# Autodesk Inventor assembly: Assembly1
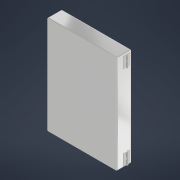
[picture p0: Inventor's stored thumbnail of the model, 180x180]
Saved by Autodesk Inventor 2022 (Build 260153000, 153)
## iProperties
Created: 2021-05-25
Part Number: Assembly1
Document SubType Name: Assembly
Designer: Albert L Tomberg
Mass: 5171.74 g
Surface Area: 5904.03 cm^2
Volume: 1915.46 cm^3
Density: 2.7 g/cm^3
Author: Albert L Tomberg
## Documents named in this file (4)
- C:\Users\Albert L Tomberg\Documents\CAD School\Assembly1.iam
- C:\Users\Albert L Tomberg\Documents\CAD School\Pocker lower half.ipt
- C:\Users\Albert L Tomberg\Documents\CAD School\Pocker higher half.ipt
- C:\Users\Albert L Tomberg\Documents\CAD School\Hinge.iam
## Components (4 placed, 3 different names)
1. Pocker lower half:1 — Mate:1, Mate:2, Mate:11, Mate:12, Mate:13
2. Pocker higher half:1 — Mate:4, Mate:6, Mate:7, Mate:8, Mate:12
3. Hinge:1 [sub-assembly] — Mate:4, Flush:1, Mate:7, Mate:11, Mate:13
4. Hinge:2 [sub-assembly] — Mate:6, Flush:1, Mate:8
## Relationships (10: Mate 9, Flush 1)
- Mate:1: Pocker lower half:1
- Mate:2: Pocker lower half:1
- Mate:4: Pocker higher half:1 ↔ Hinge:1
- Mate:6: Pocker higher half:1 ↔ Hinge:2
- Flush:1: Hinge:1 ↔ Hinge:2
- Mate:7: Pocker higher half:1 ↔ Hinge:1
- Mate:8: Pocker higher half:1 ↔ Hinge:2
- Mate:11: Pocker lower half:1 ↔ Hinge:1
- Mate:12: Pocker lower half:1 ↔ Pocker higher half:1
- Mate:13: Pocker lower half:1 ↔ Hinge:1
